# Autodesk Inventor assembly: g7_caixa_esp
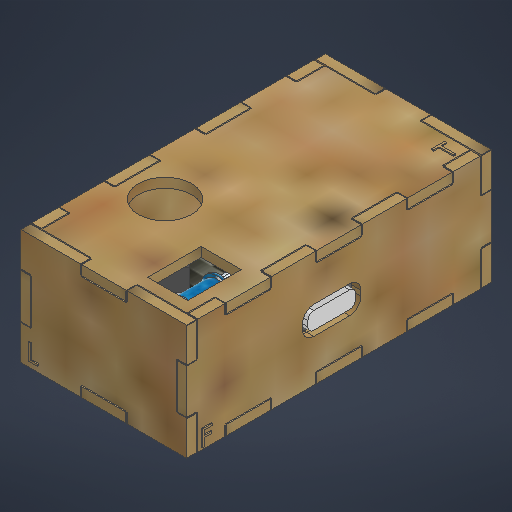
[picture p0: Inventor's stored thumbnail of the model, 512x512]
Saved by Autodesk Inventor 2026.2 (Build 302298010, 298A)
## iProperties
Created: 2026-05-20
Part Number: g7_caixa_esp
Document SubType Name: Assembly
Designer: anton
Author: anton
## Documents named in this file (15)
- C:\Users\anton\OneDrive\Documentos\FICSAE\2026.1\0.PBL.2026.1\Models\g7_caixa_esp.iam
- C:\Users\anton\OneDrive\Documentos\FICSAE\2026.1\0.PBL.2026.1\Models\ESP32_C3_SM.ipt
- C:\Users\anton\OneDrive\Documentos\FICSAE\2026.1\0.PBL.2026.1\Models\conexoes_embaixo.ipt
- C:\Users\anton\OneDrive\Documentos\FICSAE\2026.1\0.PBL.2026.1\Models\LED_RGB.ipt
- C:\Users\anton\OneDrive\Documentos\FICSAE\2026.1\0.PBL.2026.1\Models\MPU6050.ipt
- C:\Users\anton\OneDrive\Documentos\FICSAE\2026.1\0.PBL.2026.1\Models\Btn.ipt
- C:\Users\anton\OneDrive\Documentos\FICSAE\2026.1\0.PBL.2026.1\Models\base.ipt
- C:\Users\anton\OneDrive\Documentos\FICSAE\2026.1\0.PBL.2026.1\Models\caia.ipt
- C:\Users\anton\OneDrive\Documentos\FICSAE\2026.1\0.PBL.2026.1\Models\caixa_mdf.iam
- C:\Users\anton\OneDrive\Documentos\FICSAE\2026.1\0.PBL.2026.1\Models\Solid1.ipt
- C:\Users\anton\OneDrive\Documentos\FICSAE\2026.1\0.PBL.2026.1\Models\Solid2.ipt
- C:\Users\anton\OneDrive\Documentos\FICSAE\2026.1\0.PBL.2026.1\Models\Solid3.ipt
- C:\Users\anton\OneDrive\Documentos\FICSAE\2026.1\0.PBL.2026.1\Models\Solid4.ipt
- C:\Users\anton\OneDrive\Documentos\FICSAE\2026.1\0.PBL.2026.1\Models\Solid5.ipt
- C:\Users\anton\OneDrive\Documentos\FICSAE\2026.1\0.PBL.2026.1\Models\Solid6.ipt
## Components (14 placed, 14 different names)
1. ESP32_C3_SM:1 — Flush:1, Mate:1, Mate:2, Mate:3, Mate:4, Angle:1, Mate:5, Mate:6, Mate:7, Flush:2, Mate:9, Flush:3, Flush:9, Mate:14, Flush:13, Mate:16, Mate:17
2. conexoes_embaixo:1 — Flush:1, Mate:1, Mate:2, Mate:11
3. LED_RGB:1 — Mate:6, Mate:7, Flush:2
4. MPU6050:1 — Flush:9, Mate:9, Flush:3, Mate:10, Mate:12
5. Btn:1 — Mate:3, Mate:4, Angle:1, Mate:5
6. base:1 — Mate:10, Mate:11, Mate:12, Mate:13, Mate:15
7. caia:1 — Mate:13, Mate:14, Mate:15
8. Solid1:1 — Flush:23, Flush:24, Flush:25
9. Solid2:1 — Flush:10, Flush:11, Flush:12, Flush:18, Flush:19, Flush:22
10. Solid3:1 — Flush:20, Flush:21, Flush:22
11. Solid4:1 — Flush:10, Flush:11, Flush:12, Flush:13, Mate:16, Mate:17, Flush:14, Flush:15, Flush:16, Flush:17, Flush:23, Flush:25
12. Solid5:1 — Flush:14, Flush:15, Flush:16, Flush:21, Flush:24
13. Solid6:1 — Flush:17, Flush:18, Flush:19, Flush:20
14. caixa_mdf:1 [sub-assembly]
## Relationships (37: Flush 20, Mate 16, Angle 1)
- Flush:1: ESP32_C3_SM:1 ↔ conexoes_embaixo:1
- Mate:1: ESP32_C3_SM:1 ↔ conexoes_embaixo:1
- Mate:2: ESP32_C3_SM:1 ↔ conexoes_embaixo:1
- Mate:3: ESP32_C3_SM:1 ↔ Btn:1
- Mate:4: ESP32_C3_SM:1 ↔ Btn:1
- Angle:1 (45 deg): ESP32_C3_SM:1 ↔ Btn:1
- Mate:5: ESP32_C3_SM:1 ↔ Btn:1
- Mate:6 (7.5 mm): ESP32_C3_SM:1 ↔ LED_RGB:1
- Mate:7 (5 mm): ESP32_C3_SM:1 ↔ LED_RGB:1
- Flush:2 (-1 mm): ESP32_C3_SM:1 ↔ LED_RGB:1
- Flush:9: ESP32_C3_SM:1 ↔ MPU6050:1
- Mate:9 (1 mm): ESP32_C3_SM:1 ↔ MPU6050:1
- Flush:3 (-1 mm): ESP32_C3_SM:1 ↔ MPU6050:1
- Mate:10: MPU6050:1 ↔ base:1
- Mate:11: conexoes_embaixo:1 ↔ base:1
- Mate:12: MPU6050:1 ↔ base:1
- Mate:13: base:1 ↔ caia:1
- Mate:14 (1 mm): ESP32_C3_SM:1 ↔ caia:1
- Mate:15 (0.05 mm): base:1 ↔ caia:1
- Flush:10: Solid2:1 ↔ Solid4:1
- Flush:11: Solid2:1 ↔ Solid4:1
- Flush:12: Solid2:1 ↔ Solid4:1
- Flush:13: ESP32_C3_SM:1 ↔ Solid4:1
- Mate:16 (1 mm): ESP32_C3_SM:1 ↔ Solid4:1
- Mate:17 (1 mm): ESP32_C3_SM:1 ↔ Solid4:1
- Flush:14: Solid4:1 ↔ Solid5:1
- Flush:15: Solid4:1 ↔ Solid5:1
- Flush:16: Solid4:1 ↔ Solid5:1
- Flush:17: Solid4:1 ↔ Solid6:1
- Flush:18: Solid2:1 ↔ Solid6:1
- Flush:19: Solid2:1 ↔ Solid6:1
- Flush:20: Solid3:1 ↔ Solid6:1
- Flush:21: Solid3:1 ↔ Solid5:1
- Flush:22: Solid2:1 ↔ Solid3:1
- Flush:23: Solid1:1 ↔ Solid4:1
- Flush:24: Solid1:1 ↔ Solid5:1
- Flush:25: Solid1:1 ↔ Solid4:1
## Named parameters: Finish10_Area = 10.4575, Finish11_Area = 7.308, Finish12_Area = 7.308, Finish13_Area = 2.07584, Finish14_Area = 53.2697, Finish15_Area = 145.515, Finish16_Area = 145.515, Finish17_Area = 10.4575, Finish18_Area = 1.93302, Finish19_Area = 2.07584, Finish1_Area = 1.42942, Finish20_Area = 2.07584, Finish2_Area = 34.1586, Finish3_Area = 0.492052, Finish4_Area = 1.6586, Finish5_Area = 50.1397, Finish6_Area = 1.22379, Finish7_Area = 3.73795, Finish8_Area = 3.75856, Finish9_Area = 3.75856
note: some values were not read from the file. Shown as the stored number, unit unknown: "Finish10_Area", "Finish11_Area", "Finish12_Area", "Finish13_Area", "Finish14_Area", "Finish15_Area", "Finish16_Area", "Finish17_Area", "Finish18_Area", "Finish19_Area", "Finish1_Area", "Finish20_Area", "Finish2_Area", "Finish3_Area", "Finish4_Area", "Finish5_Area", "Finish6_Area", "Finish7_Area", "Finish8_Area", "Finish9_Area".
